# Autodesk Inventor assembly: SM_XA01
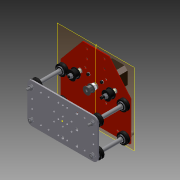
[picture p0: Inventor's stored thumbnail of the model, 180x180]
Saved by Autodesk Inventor 2013 (Build 170138000, 138)
## iProperties
Created: 2012-05-01
Part Number: SM_XA01
Document SubType Name: Assembly
Designer: ERF
Description: X Axis Motor Mount Plate
Stock Number: SM_XA01
Author: ERF
Title: X Axis Motor Mount Plate Assembly
## Documents named in this file (17)
- C:\Users\Brett\Documents\GitHub\BigOko\Assemblies\SM-XA01.iam
- C:\Users\Brett\Documents\GitHub\BigOko\Parts\SM-H04.ipt
- C:\Users\Brett\Documents\GitHub\BigOko\Parts\SM-H01.ipt
- C:\Users\Brett\Documents\GitHub\BigOko\Parts\MSK01-04.ipt
- C:\Users\Brett\Documents\GitHub\BigOko\Parts\SM-H08.ipt
- C:\Users\Brett\Documents\GitHub\BigOko\Parts\SM-S01.ipt
- C:\Users\Brett\Documents\GitHub\BigOko\Parts\MSK01-09.ipt
- C:\Users\Brett\Documents\GitHub\BigOko\Parts\SM-E01.ipt
- C:\Users\Brett\Documents\GitHub\BigOko\Parts\SM-H03.ipt
- C:\Users\Brett\Documents\GitHub\BigOko\Parts\SM-H14.ipt
- C:\Users\Brett\Documents\GitHub\BigOko\Parts\SM-H15.ipt
- C:\Users\Brett\Documents\GitHub\BigOko\Assemblies\MSK01-06A.iam
- C:\Users\Brett\Documents\GitHub\BigOko\Assemblies\MSK01-05A.iam
- C:\Users\Brett\Documents\GitHub\BigOko\bb_parts\Imported Components\shc_90mm\shc_90mm.ipt
- C:\Users\Brett\Documents\GitHub\BigOko\Assemblies\SM-ZA01.iam
- C:\Users\Brett\Documents\GitHub\BigOko\bb_parts\Imported Components\standoff_m5_45mm\standoff_m5_45mm.ipt
- C:\Users\Brett\Documents\GitHub\BigOko\Parts\MSK01-05A.ipt
## Components (82 placed, 15 different names)
1. standoff_m5_45mm:1
2. standoff_m5_45mm:2
3. standoff_m5_45mm:3
4. standoff_m5_45mm:4
5. SM-H03:27
6. SM-H03:28
7. SM-H03:29
8. SM-H03:30
9. SM-H03:31
10. SM-H03:32
11. SM-H03:33
12. SM-H03:34
13. MSK01-05A:9
14. MSK01-05A:10
15. MSK01-05A:11
16. MSK01-05A:12
17. SM-H03:35
18. SM-H03:36 — Insert:117, Insert:119
19. SM-H03:37 — Insert:113
20. SM-H03:38
21. SM-H03:39
22. SM-H03:40 — Insert:111
23. SM-H03:41 — Insert:116, Insert:118
24. SM-H03:42 — Insert:115
25. SM-ZA01:1 [sub-assembly] — Insert:115, Insert:116, Insert:117
26. SM-H04:1 — Insert:55
27. SM-H01:1 — Insert:26, Insert:28
28. SM-H04:2 — Insert:54
29. MSK01-04:1 — Insert:5, Insert:8
30. SM-H01:2 — Insert:25, Insert:27
31. MSK01-04:2 — Insert:6, Insert:7
32. SM-H08:1 — Insert:9
33. SM-H08:2 — Insert:10
34. SM-S01:1 — Insert:7, Insert:8, Insert:11, Insert:12, Insert:13, Insert:14, Insert:16, Insert:17, Insert:37, Mate:4, Mate:5, Mate:6, Insert:56, Angle:1, Insert:61, Insert:62, Insert:63, Insert:64, Insert:114
35. MSK01-06A:3 [sub-assembly] — Insert:66, Insert:67
36. MSK01-06A:4 [sub-assembly] — Insert:68, Insert:69
37. MSK01-09:1 — Insert:65
38. MSK01-05A:5 [sub-assembly] — Insert:70, Insert:71
39. MSK01-05A:6 [sub-assembly] — Insert:76, Insert:77
40. MSK01-05A:7 [sub-assembly] — Insert:74, Insert:75
41. MSK01-05A:8 [sub-assembly] — Insert:72, Insert:73
42. SM-E01:1 — Insert:56, Angle:1, Insert:65
43. SM-H03:2 — Insert:5, Insert:78
44. SM-H03:3 — Insert:13, Insert:80
45. SM-H03:4 — Insert:14, Insert:79
46. SM-H03:5 — Insert:6, Insert:81
47. SM-H03:6 — Insert:10, Insert:12
48. SM-H03:7 — Insert:9, Insert:11
49. SM-H03:8 — Insert:76, Insert:85
50. SM-H03:9 — Insert:70, Insert:84
51. SM-H03:10 — Insert:16, Insert:25
52. SM-H03:11 — Insert:17, Insert:26
53. SM-H03:12 — Insert:74, Insert:82
54. SM-H03:13 — Insert:72, Insert:83
55. SM-H03:14 — Insert:27, Insert:68
56. SM-H03:15 — Insert:28, Insert:66
57. SM-H03:16 — Insert:55, Insert:67
58. SM-H03:17 — Insert:54, Insert:69
59. SM-H03:18 — Insert:84
60. SM-H03:19 — Insert:85
61. SM-H03:20 — Insert:83
62. SM-H03:21 — Insert:82
63. SM-H03:22 — Mate:5, Insert:75
64. SM-H03:23 — Mate:6, Insert:73, Insert:114
65. SM-H03:25 — Mate:4, Insert:77
66. SM-H03:26 — Insert:37, Insert:71
67. SM-H15:2 — Insert:57, Insert:64
68. SM-H14:2 — Insert:57
69. SM-H15:3 — Insert:58, Insert:62
70. SM-H14:3 — Insert:58
71. SM-H15:4 — Insert:60, Insert:63
72. SM-H14:4 — Insert:60
73. SM-H15:5 — Insert:59, Insert:61
74. SM-H14:5 — Insert:59
75. shc_90mm:1 — Insert:78
76. shc_90mm:2 — Insert:79
77. shc_90mm:3 — Insert:81
78. shc_90mm:4 — Insert:80
79. SM-H04:3 — Insert:111
80. SM-H04:4 — Insert:118
81. SM-H04:5 — Insert:113
82. SM-H04:6 — Insert:119
## Relationships (84: Insert 80, Mate 3, Angle 1)
- Insert:5: MSK01-04:1 ↔ SM-H03:2
- Insert:6: MSK01-04:2 ↔ SM-H03:5
- Insert:7: MSK01-04:2 ↔ SM-S01:1
- Insert:8: MSK01-04:1 ↔ SM-S01:1
- Insert:9: SM-H08:1 ↔ SM-H03:7
- Insert:10: SM-H08:2 ↔ SM-H03:6
- Insert:11: SM-S01:1 ↔ SM-H03:7
- Insert:12: SM-S01:1 ↔ SM-H03:6
- Insert:13: SM-S01:1 ↔ SM-H03:3
- Insert:14: SM-S01:1 ↔ SM-H03:4
- Insert:16: SM-S01:1 ↔ SM-H03:10
- Insert:17: SM-S01:1 ↔ SM-H03:11
- Insert:25: SM-H01:2 ↔ SM-H03:10
- Insert:26: SM-H01:1 ↔ SM-H03:11
- Insert:27: SM-H01:2 ↔ SM-H03:14
- Insert:28: SM-H01:1 ↔ SM-H03:15
- Insert:37: SM-S01:1 ↔ SM-H03:26
- Mate:4: SM-S01:1 ↔ SM-H03:25
- Mate:5: SM-S01:1 ↔ SM-H03:22
- Mate:6: SM-S01:1 ↔ SM-H03:23
- Insert:54: SM-H04:2 ↔ SM-H03:17
- Insert:55: SM-H04:1 ↔ SM-H03:16
- Insert:56: SM-S01:1 ↔ SM-E01:1
- Angle:1 (0 deg): SM-S01:1 ↔ SM-E01:1
- Insert:57: SM-H15:2 ↔ SM-H14:2
- Insert:58: SM-H15:3 ↔ SM-H14:3
- Insert:59: SM-H15:5 ↔ SM-H14:5
- Insert:60: SM-H15:4 ↔ SM-H14:4
- Insert:61: SM-S01:1 ↔ SM-H15:5
- Insert:62: SM-S01:1 ↔ SM-H15:3
- Insert:63: SM-S01:1 ↔ SM-H15:4
- Insert:64: SM-S01:1 ↔ SM-H15:2
- Insert:65 (5.08 mm): MSK01-09:1 ↔ SM-E01:1
- Insert:66: MSK01-06A:3 ↔ SM-H03:15
- Insert:67: MSK01-06A:3 ↔ SM-H03:16
- Insert:68: MSK01-06A:4 ↔ SM-H03:14
- Insert:69: MSK01-06A:4 ↔ SM-H03:17
- Insert:70: MSK01-05A:5 ↔ SM-H03:9
- Insert:71: MSK01-05A:5 ↔ SM-H03:26
- Insert:72: MSK01-05A:8 ↔ SM-H03:13
- Insert:73: MSK01-05A:8 ↔ SM-H03:23
- Insert:74: MSK01-05A:7 ↔ SM-H03:12
- Insert:75: MSK01-05A:7 ↔ SM-H03:22
- Insert:76: MSK01-05A:6 ↔ SM-H03:8
- Insert:77: MSK01-05A:6 ↔ SM-H03:25
- Insert:78: SM-H03:2 ↔ shc_90mm:1
- Insert:79: SM-H03:4 ↔ shc_90mm:2
- Insert:80: SM-H03:3 ↔ shc_90mm:4
- Insert:81: SM-H03:5 ↔ shc_90mm:3
- Insert:82: SM-H03:12 ↔ SM-H03:21
- Insert:83: SM-H03:13 ↔ SM-H03:20
- Insert:84: SM-H03:9 ↔ SM-H03:18
- Insert:85: SM-H03:8 ↔ SM-H03:19
- [Insert]: standoff_m5_45mm:1 ↔ SM-H03:21
- [Insert]: standoff_m5_45mm:2 ↔ SM-H03:20
- [Insert]: standoff_m5_45mm:3 ↔ SM-H03:18
- [Insert]: standoff_m5_45mm:4 ↔ SM-H03:19
- [Insert]: standoff_m5_45mm:2 ↔ SM-H03:27
- [Insert]: SM-H03:27 ↔ SM-H03:30
- [Insert]: standoff_m5_45mm:1 ↔ SM-H03:29
- [Insert]: SM-H03:28 ↔ SM-H03:29
- [Insert]: standoff_m5_45mm:3 ↔ SM-H03:34
- [Insert]: SM-H03:33 ↔ SM-H03:34
- [Insert]: standoff_m5_45mm:4 ↔ SM-H03:32
- [Insert]: SM-H03:31 ↔ SM-H03:32
- [Insert]: SM-H03:33 ↔ MSK01-05A:12
- [Insert]: SM-H03:31 ↔ MSK01-05A:11
- [Insert]: SM-H03:30 ↔ MSK01-05A:10
- [Insert]: SM-H03:29 ↔ MSK01-05A:9
- [Insert]: MSK01-05A:12 ↔ SM-H03:42
- [Insert]: MSK01-05A:11 ↔ SM-H03:35
- [Insert]: MSK01-05A:10 ↔ SM-H03:38
- [Insert]: MSK01-05A:9 ↔ SM-H03:39
- [Insert]: SM-H03:38 ↔ SM-ZA01:1
- [Insert]: SM-H03:37 ↔ SM-ZA01:1
- [Insert]: SM-H03:40 ↔ SM-ZA01:1
- Insert:111: SM-H03:40 ↔ SM-H04:3
- Insert:113: SM-H03:37 ↔ SM-H04:5
- Insert:114: SM-S01:1 ↔ SM-H03:23
- Insert:115: SM-H03:42 ↔ SM-ZA01:1
- Insert:116: SM-H03:41 ↔ SM-ZA01:1
- Insert:117: SM-H03:36 ↔ SM-ZA01:1
- Insert:118: SM-H03:41 ↔ SM-H04:4
- Insert:119: SM-H03:36 ↔ SM-H04:6
## Named parameters: d103_d15 = 0 mm, d104_d16 = 0 mm, d109_d24 = 0 mm, d110_d25 = 0 mm, d111_d26 = 0 mm, d112_d27 = 0 mm, d116_d4 = 0 mm, d117_d5 = 0 mm, d118_d6 = 0 mm, d119_d7 = 0 mm, d120_d8 = 0 mm, d121_d9 = 0 mm, d122_d10 = 0 mm, d123_d11 = 0 mm, d124_d12 = 0 mm, d125_d13 = 0 mm
